# Autodesk Inventor assembly: GeneratorPlateAssembly
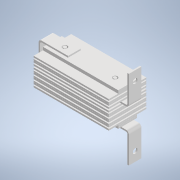
[picture p0: Inventor's stored thumbnail of the model, 180x180]
Saved by Autodesk Inventor 2020 (Build 240168000, 168)
## iProperties
Created: 2020-01-01
Part Number: GeneratorPlateAssembly
Document SubType Name: Assembly
Designer: ellio
Author: ellio
## Documents named in this file (7)
- E:\TEMP BACKUP FOR MW\TEMPDOCS\HHO PARTS\GeneratorPlateAssembly.iam
- E:\TEMP BACKUP FOR MW\TEMPDOCS\HHO PARTS\plates\6x3.ipt
- E:\TEMP BACKUP FOR MW\TEMPDOCS\HHO PARTS\Nylon Rod.ipt
- E:\TEMP BACKUP FOR MW\TEMPDOCS\HHO PARTS\plates\4.5x1 BENT.ipt
- E:\TEMP BACKUP FOR MW\TEMPDOCS\HHO PARTS\plates\6x1.5.ipt
- E:\TEMP BACKUP FOR MW\TEMPDOCS\HHO PARTS\plates\6x1 BENT.ipt
- E:\TEMP BACKUP FOR MW\TEMPDOCS\HHO PARTS\Nylon Rod - Trimmed.ipt
## Components (23 placed, 6 different names)
1. 6x3:1 — Insert:1, Insert:2, Mate:1, Flush:1, Flush:2, Flush:3, Flush:4, Mate:11, Flush:15
2. 6x3:2 — Mate:1, Flush:1, Flush:2, Mate:2
3. 6x3:3 — Mate:2, Flush:3, Flush:4, Mate:3, Flush:5, Flush:6
4. 6x3:4 — Mate:3, Flush:5, Flush:6, Mate:4, Flush:7, Flush:8
5. 6x3:5 — Mate:5, Flush:9, Flush:10, Mate:6, Flush:11, Flush:12
6. 6x3:6 — Mate:7, Flush:13, Flush:14, Mate:8, Flush:18, Flush:19
7. 6x3:7 — Mate:6, Flush:11, Flush:12, Mate:7, Flush:13, Flush:14
8. 6x3:8 — Mate:4, Flush:7, Flush:8, Mate:5, Flush:9, Flush:10
9. Nylon Rod:1 — Insert:1, Mate:23, Mate:25
10. Nylon Rod:2 — Insert:2, Mate:9, Mate:10, Mate:12, Mate:15
11. 4.5x1 BENT:1 — Mate:8, Mate:9, Mate:10, Mate:18
12. 6x1.5:1 — Mate:11, Flush:15, Mate:12, Mate:13, Flush:16, Flush:17
13. 6x1.5:2 — Mate:13, Flush:16, Flush:17, Mate:14
14. 4.5x1 BENT:2 — Mate:14, Mate:15
15. 6x3:9 — Mate:18, Flush:18, Flush:19, Mate:19, Flush:20, Flush:21
16. 6x3:10 — Mate:20, Flush:22, Flush:23, Mate:21, Flush:24, Flush:25
17. 6x3:11 — Mate:19, Flush:20, Flush:21, Mate:20, Flush:22, Flush:23
18. 6x3:12 — Mate:21, Flush:24, Flush:25, Mate:22, Flush:26
19. 6x1.5:3 — Mate:22, Mate:23, Flush:26, Mate:24, Flush:27, Flush:28
20. 6x1.5:4 — Mate:24, Flush:27, Flush:28, Mate:26, Mate:28, Flush:30
21. 6x1 BENT:1 — Mate:25, Mate:26, Mate:27, Flush:29
22. Nylon Rod - Trimmed:1 — Mate:27, Flush:29
23. Nylon Rod - Trimmed:2 — Mate:28, Flush:30
## Relationships (58: Flush 30, Mate 26, Insert 2)
- Insert:1 (-10.16 mm): 6x3:1 ↔ Nylon Rod:1
- Insert:2 (-10.16 mm): 6x3:1 ↔ Nylon Rod:2
- Mate:1 (2.54 mm): 6x3:1 ↔ 6x3:2
- Flush:1: 6x3:1 ↔ 6x3:2
- Flush:2: 6x3:1 ↔ 6x3:2
- Mate:2 (0.127 mm): 6x3:2 ↔ 6x3:3
- Flush:3: 6x3:1 ↔ 6x3:3
- Flush:4: 6x3:1 ↔ 6x3:3
- Mate:3 (2.54 mm): 6x3:3 ↔ 6x3:4
- Flush:5: 6x3:3 ↔ 6x3:4
- Flush:6: 6x3:3 ↔ 6x3:4
- Mate:4 (0.127 mm): 6x3:4 ↔ 6x3:8
- Flush:7: 6x3:4 ↔ 6x3:8
- Flush:8: 6x3:4 ↔ 6x3:8
- Mate:5 (2.54 mm): 6x3:5 ↔ 6x3:8
- Flush:9: 6x3:5 ↔ 6x3:8
- Flush:10: 6x3:5 ↔ 6x3:8
- Mate:6 (0.127 mm): 6x3:5 ↔ 6x3:7
- Flush:11: 6x3:5 ↔ 6x3:7
- Flush:12: 6x3:5 ↔ 6x3:7
- Mate:7 (2.54 mm): 6x3:6 ↔ 6x3:7
- Flush:13: 6x3:6 ↔ 6x3:7
- Flush:14: 6x3:6 ↔ 6x3:7
- Mate:8: 6x3:6 ↔ 4.5x1 BENT:1
- Mate:9: Nylon Rod:2 ↔ 4.5x1 BENT:1
- Mate:10: Nylon Rod:2 ↔ 4.5x1 BENT:1
- Mate:11 (0.127 mm): 6x3:1 ↔ 6x1.5:1
- Flush:15: 6x3:1 ↔ 6x1.5:1
- Mate:12: Nylon Rod:2 ↔ 6x1.5:1
- Mate:13 (0.127 mm): 6x1.5:1 ↔ 6x1.5:2
- Flush:16: 6x1.5:1 ↔ 6x1.5:2
- Flush:17: 6x1.5:1 ↔ 6x1.5:2
- Mate:14: 6x1.5:2 ↔ 4.5x1 BENT:2
- Mate:15: Nylon Rod:2 ↔ 4.5x1 BENT:2
- Mate:18: 4.5x1 BENT:1 ↔ 6x3:9
- Flush:18: 6x3:6 ↔ 6x3:9
- Flush:19: 6x3:6 ↔ 6x3:9
- Mate:19 (2.54 mm): 6x3:9 ↔ 6x3:11
- Flush:20: 6x3:9 ↔ 6x3:11
- Flush:21: 6x3:9 ↔ 6x3:11
- Mate:20 (0.127 mm): 6x3:10 ↔ 6x3:11
- Flush:22: 6x3:10 ↔ 6x3:11
- Flush:23: 6x3:10 ↔ 6x3:11
- Mate:21 (2.54 mm): 6x3:10 ↔ 6x3:12
- Flush:24: 6x3:10 ↔ 6x3:12
- Flush:25: 6x3:10 ↔ 6x3:12
- Mate:22: 6x3:12 ↔ 6x1.5:3
- Mate:23: Nylon Rod:1 ↔ 6x1.5:3
- Flush:26: 6x3:12 ↔ 6x1.5:3
- Mate:24: 6x1.5:3 ↔ 6x1.5:4
- Flush:27: 6x1.5:3 ↔ 6x1.5:4
- Flush:28: 6x1.5:3 ↔ 6x1.5:4
- Mate:25: Nylon Rod:1 ↔ 6x1 BENT:1
- Mate:26: 6x1.5:4 ↔ 6x1 BENT:1
- Mate:27: 6x1 BENT:1 ↔ Nylon Rod - Trimmed:1
- Flush:29: 6x1 BENT:1 ↔ Nylon Rod - Trimmed:1
- Mate:28: 6x1.5:4 ↔ Nylon Rod - Trimmed:2
- Flush:30: 6x1.5:4 ↔ Nylon Rod - Trimmed:2
